# Autodesk Inventor assembly: Robot B
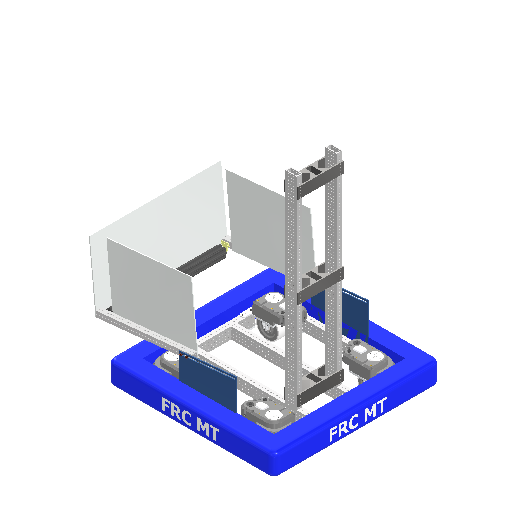
[picture p0: Inventor's stored thumbnail of the model, 512x512]
Saved by Autodesk Inventor 2025.3 (Build 293356000, 356)
## iProperties
Created: 2026-05-13
Part Number: Robot B
Document SubType Name: Assembly
Designer: djair.oliveira
Author: djair.oliveira
## Documents named in this file (5)
- C:\Users\djair.oliveira\Documents\GitHub\MT_2026\CAD\Model B\Robot B.iam
- C:\Users\djair.oliveira\Documents\GitHub\MT_2026\CAD\Model B\Chassi\Chassi.iam
- C:\Users\djair.oliveira\Documents\GitHub\MT_2026\CAD\Model B\Elevador\Elevador.iam
- C:\Users\djair.oliveira\Documents\GitHub\MT_2026\CAD\Model B\Intake\Intake.iam
- C:\Users\djair.oliveira\Documents\GitHub\MT_2026\CAD\Model B\Bumper.ipt
## Components (4 placed, 4 different names)
1. Chassi:1 [sub-assembly] — Coincidente:1, Alinhado:1, Alinhado:4, Coincidente:3, Coincidente:4, Coincidente:5, Tangente:1, Coincidente:7, Coincidente:8, Coincidente:9, Alinhado:5
2. Elevador:1 [sub-assembly] — Coincidente:1, Alinhado:1, Alinhado:4, Coincidente:6
3. Intake:1 [sub-assembly] — Coincidente:3, Coincidente:4, Coincidente:5
4. Bumper:1 — Coincidente:8, Coincidente:9, Alinhado:5
## Relationships (12: Mate 8, Flush 3, Tangent 1)
- Coincidente:1 [Mate]: Chassi:1 ↔ Elevador:1
- Alinhado:1 [Flush]: Chassi:1 ↔ Elevador:1
- Alinhado:4 [Flush] (88.9 mm): Chassi:1 ↔ Elevador:1
- Coincidente:3 [Mate]: Chassi:1 ↔ Intake:1
- Coincidente:4 [Mate]: Chassi:1 ↔ Intake:1
- Coincidente:5 [Mate]: Chassi:1 ↔ Intake:1
- Tangente:1: Chassi:1
- Coincidente:6 [Mate] (76.2 mm): Elevador:1
- Coincidente:7 [Mate] (-292.1 mm): Chassi:1
- Coincidente:8 [Mate]: Chassi:1 ↔ Bumper:1
- Coincidente:9 [Mate]: Chassi:1 ↔ Bumper:1
- Alinhado:5 [Flush]: Chassi:1 ↔ Bumper:1
